# Autodesk Inventor assembly: Gripper
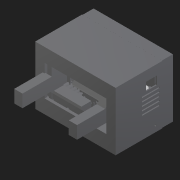
[picture p0: Inventor's stored thumbnail of the model, 180x180]
Saved by Autodesk Inventor 2017 (Build 210142000, 142)
## iProperties
Created: 2018-10-23
Part Number: Gripper
Document SubType Name: Assembly
Designer: Dell
Author: Dell
## Documents named in this file (8)
- C:\Users\Dell\Documents\GitHub\tr2\Gripper 1.1\Gripper 1.1.iam
- C:\Users\Dell\Documents\GitHub\tr2\Gripper 1.1\Gripper\Design Accelerator\Spur Gears1.iam
- C:\Users\Dell\Documents\GitHub\tr2\Gripper 1.1\GA04.ipt
- C:\Users\Dell\Documents\GitHub\tr2\Gripper 1.1\GA01b.ipt
- C:\Users\Dell\Documents\GitHub\tr2\Gripper 1.1\GA06.ipt
- C:\Users\Dell\Documents\GitHub\tr2\Gripper 1.1\GA07.ipt
- C:\Users\Dell\Documents\GitHub\tr2\Gripper 1.1\GA08.ipt
- C:\Users\Dell\Documents\GitHub\tr2\Gripper 1.1\Motor.ipt
## Components (9 placed, 7 different names)
1. GA01b:1 — Mate:28, Mate:29, Mate:30, Mate:44, Mate:52, Mate:54, Mate:55, Mate:56, Mate:57, Mate:60, Mate:61, Mate:63, Mate:65, Mate:66, Mate:70, Mate:71
2. GA04:3 — Mate:28, Rotation/Translation:3, Mate:44, Flush:1, Mate:67, Mate:68, Mate:69
3. GA04:4 — Mate:29, Mate:30, Rotation/Translation:4, Mate:45, Mate:46, Mate:47
4. Spur Gears:2 [sub-assembly] — Rotation/Translation:3, Rotation/Translation:4, Mate:64, Flush:1
5. GA06:1 — Mate:60, Mate:61, Mate:70, Mate:71
6. GA07:1 — Mate:45, Mate:46, Mate:47, Mate:54
7. GA08:1 — Mate:55, Mate:56, Mate:57
8. Motor:1 — Mate:63, Mate:64, Mate:65, Mate:66
9. GA07:2 — Mate:67, Mate:68, Mate:69
## Relationships (26: Mate 23, RelateRotateTranslate 2, Flush 1)
- Mate:28: GA01b:1 ↔ GA04:3
- Mate:29: GA01b:1 ↔ GA04:4
- Mate:30: GA01b:1 ↔ GA04:4
- Rotation/Translation:3 [RelateRotateTranslate] (131 mm): GA04:3 ↔ Spur Gears:2
- Rotation/Translation:4 [RelateRotateTranslate] (131 mm): GA04:4 ↔ Spur Gears:2
- Mate:44: GA01b:1 ↔ GA04:3
- Mate:45: GA04:4 ↔ GA07:1
- Mate:46: GA04:4 ↔ GA07:1
- Mate:47: GA04:4 ↔ GA07:1
- Mate:52: GA01b:1
- Mate:54: GA01b:1 ↔ GA07:1
- Mate:55: GA01b:1 ↔ GA08:1
- Mate:56: GA01b:1 ↔ GA08:1
- Mate:57: GA01b:1 ↔ GA08:1
- Mate:60: GA01b:1 ↔ GA06:1
- Mate:61: GA01b:1 ↔ GA06:1
- Mate:63: GA01b:1 ↔ Motor:1
- Mate:64: Spur Gears:2 ↔ Motor:1
- Mate:65: GA01b:1 ↔ Motor:1
- Mate:66: GA01b:1 ↔ Motor:1
- Flush:1: GA04:3 ↔ Spur Gears:2
- Mate:67: GA04:3 ↔ GA07:2
- Mate:68: GA04:3 ↔ GA07:2
- Mate:69: GA04:3 ↔ GA07:2
- Mate:70 (2 mm): GA01b:1 ↔ GA06:1
- Mate:71: GA01b:1 ↔ GA06:1
